# Autodesk Inventor assembly: switchback
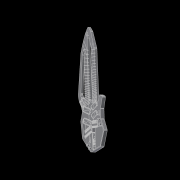
[picture p0: Inventor's stored thumbnail of the model, 180x180]
Saved by Autodesk Inventor 2020 (Build 240168000, 168)
## iProperties
Created: 2020-01-02
Part Number: switchback
Document SubType Name: Assembly
Designer: valer
Author: valer
## Documents named in this file (17)
- C:\Users\valer\Desktop\switchback\switchback.iam
- C:\Users\valer\Desktop\switchback\switchback.ipt
- C:\Users\valer\Desktop\switchback\strandberg-headless-tuner.ipt
- C:\Users\valer\Desktop\switchback\fishman-modern6.ipt
- C:\Users\valer\Desktop\switchback\fishman-modern8.ipt
- C:\Users\valer\Desktop\switchback\fishman-pot.ipt
- C:\Users\valer\Desktop\switchback\fishman-switch.ipt
- C:\Users\valer\Desktop\switchback\fishman-battery.ipt
- C:\Users\valer\Desktop\switchback\switchback-secondary-cover.ipt
- C:\Users\valer\Desktop\switchback\switchback-primary-cover.ipt
- C:\Users\valer\Desktop\switchback\fishman-jack.ipt
- C:\Users\valer\Desktop\switchback\switchback-pickup-cover-8.ipt
- C:\Users\valer\Desktop\switchback\switchback-pickup-cover-6.ipt
- C:\Users\valer\Desktop\switchback\switchback-logo-01.ipt
- C:\Users\valer\Desktop\switchback\arduino.ipt
- C:\Users\valer\Desktop\switchback\oscilloscope-screen.ipt
- C:\Users\valer\Desktop\switchback\switchback-osc-cover.ipt
## Components (38 placed, 16 different names)
1. switchback:1 — Mate:1, Mate:2, Tangent:1, Mate:4, Mate:5, Tangent:2, Mate:6, Mate:7, Tangent:3, Mate:8, Mate:9, Tangent:4, Mate:10, Mate:11, Tangent:5, Mate:12, Mate:13, Tangent:6, Mate:14, Mate:15, Tangent:7, Mate:16, Mate:17, Tangent:8, Mate:28, Mate:29, Tangent:14, Mate:42, Mate:43, Tangent:15, Mate:44, Mate:45, Tangent:16, Mate:46, Mate:47, Tangent:17, Mate:48, Mate:49, Tangent:18, Mate:50, Mate:51, Tangent:19, Mate:52, Mate:53, Mate:54, Mate:55, Mate:56, Mate:57, Mate:58, Mate:59, Mate:60, Mate:61, Mate:62, Mate:63, Mate:66, Mate:67, Mate:68, Mate:69, Mate:70, Mate:71, Mate:72, Mate:73, Angle:1, Angle:2, Angle:3, Angle:4, Mate:74, Mate:75, Mate:76, Mate:77, Mate:78, Mate:79, Mate:80, Mate:81, Mate:82, Mate:83, Mate:104, Mate:105, Mate:106, Mate:107, Mate:108, Mate:109, Flush:1, Mate:110, Mate:111, Mate:112, Mate:113, Mate:114, Mate:121, Mate:122
2. strandberg-headless-tuner:1 — Mate:1, Mate:2, Tangent:1
3. strandberg-headless-tuner:2 — Mate:4, Mate:5, Tangent:2
4. strandberg-headless-tuner:3 — Mate:6, Mate:7, Tangent:3
5. strandberg-headless-tuner:4 — Mate:10, Mate:11, Tangent:5
6. strandberg-headless-tuner:5 — Mate:12, Mate:13, Tangent:6
7. strandberg-headless-tuner:6 — Mate:8, Mate:9, Tangent:4
8. strandberg-headless-tuner:8 — Mate:14, Mate:15, Tangent:7
9. strandberg-headless-tuner:9 — Mate:16, Mate:17, Tangent:8
10. strandberg-headless-tuner:15 — Mate:28, Mate:29, Tangent:14
11. strandberg-headless-tuner:16 — Mate:46, Mate:47, Tangent:17
12. strandberg-headless-tuner:17 — Mate:48, Mate:49, Tangent:18
13. strandberg-headless-tuner:18 — Mate:42, Mate:43, Tangent:15
14. strandberg-headless-tuner:19 — Mate:44, Mate:45, Tangent:16
15. strandberg-headless-tuner:20 — Mate:50, Mate:51, Tangent:19
16. fishman-modern6:1 — Mate:52, Mate:53, Mate:54, Mate:101, Mate:102, Mate:103
17. fishman-modern6:2 — Mate:55, Mate:56, Mate:57, Mate:98, Mate:99, Mate:100
18. fishman-modern8:1 — Mate:61, Mate:62, Mate:63, Mate:92, Mate:95, Mate:96, Mate:97
19. fishman-modern8:2 — Mate:58, Mate:59, Mate:60, Mate:93, Mate:94
20. fishman-pot:1 — Mate:72, Mate:73, Angle:4
21. fishman-pot:2 — Mate:70, Mate:71, Angle:3
22. fishman-pot:4 — Mate:66, Mate:67, Angle:2
23. fishman-pot:5 — Mate:68, Mate:69, Angle:1
24. fishman-switch:1 — Mate:77, Mate:78, Mate:79
25. fishman-switch:2 — Mate:74, Mate:75, Mate:76
26. fishman-battery:1 — Mate:80, Mate:115, Mate:116, Angle:5
27. switchback-secondary-cover:1 — Mate:81, Mate:82, Mate:83
28. switchback-primary-cover:1 — Mate:115, Mate:116, Angle:5, Mate:117, Mate:118, Mate:119, Mate:120, Mate:121, Mate:122
29. fishman-jack:1 — Mate:118, Mate:119
30. fishman-jack:2 — Mate:117, Mate:120
31. switchback-pickup-cover-8:1 — Mate:92, Mate:93, Mate:94
32. switchback-pickup-cover-8:2 — Mate:95, Mate:96, Mate:97
33. switchback-pickup-cover-6:2 — Mate:98, Mate:99, Mate:100
34. switchback-pickup-cover-6:3 — Mate:101, Mate:102, Mate:103
35. switchback-logo-01:1 — Mate:104, Mate:105, Mate:106
36. arduino:1 — Mate:107, Mate:108, Mate:109
37. OscilloscopeScreen:1 — Flush:1, Mate:110, Mate:111
38. switchback-osc-cover:1 — Mate:112, Mate:113, Mate:114
## Relationships (109: Mate 89, Tangent 14, Angle 5, Flush 1)
- Mate:1: switchback:1 ↔ strandberg-headless-tuner:1
- Mate:2: switchback:1 ↔ strandberg-headless-tuner:1
- Tangent:1: switchback:1 ↔ strandberg-headless-tuner:1
- Mate:4: switchback:1 ↔ strandberg-headless-tuner:2
- Mate:5: switchback:1 ↔ strandberg-headless-tuner:2
- Tangent:2: switchback:1 ↔ strandberg-headless-tuner:2
- Mate:6: switchback:1 ↔ strandberg-headless-tuner:3
- Mate:7: switchback:1 ↔ strandberg-headless-tuner:3
- Tangent:3: switchback:1 ↔ strandberg-headless-tuner:3
- Mate:8: switchback:1 ↔ strandberg-headless-tuner:6
- Mate:9: switchback:1 ↔ strandberg-headless-tuner:6
- Tangent:4: switchback:1 ↔ strandberg-headless-tuner:6
- Mate:10: switchback:1 ↔ strandberg-headless-tuner:4
- Mate:11: switchback:1 ↔ strandberg-headless-tuner:4
- Tangent:5: switchback:1 ↔ strandberg-headless-tuner:4
- Mate:12: switchback:1 ↔ strandberg-headless-tuner:5
- Mate:13: switchback:1 ↔ strandberg-headless-tuner:5
- Tangent:6: switchback:1 ↔ strandberg-headless-tuner:5
- Mate:14: switchback:1 ↔ strandberg-headless-tuner:8
- Mate:15: switchback:1 ↔ strandberg-headless-tuner:8
- Tangent:7: switchback:1 ↔ strandberg-headless-tuner:8
- Mate:16: switchback:1 ↔ strandberg-headless-tuner:9
- Mate:17: switchback:1 ↔ strandberg-headless-tuner:9
- Tangent:8: switchback:1 ↔ strandberg-headless-tuner:9
- Mate:28: switchback:1 ↔ strandberg-headless-tuner:15
- Mate:29: switchback:1 ↔ strandberg-headless-tuner:15
- Tangent:14: switchback:1 ↔ strandberg-headless-tuner:15
- Mate:42: switchback:1 ↔ strandberg-headless-tuner:18
- Mate:43: switchback:1 ↔ strandberg-headless-tuner:18
- Tangent:15: switchback:1 ↔ strandberg-headless-tuner:18
- Mate:44: switchback:1 ↔ strandberg-headless-tuner:19
- Mate:45: switchback:1 ↔ strandberg-headless-tuner:19
- Tangent:16: switchback:1 ↔ strandberg-headless-tuner:19
- Mate:46: switchback:1 ↔ strandberg-headless-tuner:16
- Mate:47: switchback:1 ↔ strandberg-headless-tuner:16
- Tangent:17: switchback:1 ↔ strandberg-headless-tuner:16
- Mate:48: switchback:1 ↔ strandberg-headless-tuner:17
- Mate:49: switchback:1 ↔ strandberg-headless-tuner:17
- Tangent:18: switchback:1 ↔ strandberg-headless-tuner:17
- Mate:50: switchback:1 ↔ strandberg-headless-tuner:20
- Mate:51: switchback:1 ↔ strandberg-headless-tuner:20
- Tangent:19: switchback:1 ↔ strandberg-headless-tuner:20
- Mate:52: switchback:1 ↔ fishman-modern6:1
- Mate:53: switchback:1 ↔ fishman-modern6:1
- Mate:54: switchback:1 ↔ fishman-modern6:1
- Mate:55: switchback:1 ↔ fishman-modern6:2
- Mate:56: switchback:1 ↔ fishman-modern6:2
- Mate:57: switchback:1 ↔ fishman-modern6:2
- Mate:58: switchback:1 ↔ fishman-modern8:2
- Mate:59: switchback:1 ↔ fishman-modern8:2
- Mate:60: switchback:1 ↔ fishman-modern8:2
- Mate:61: switchback:1 ↔ fishman-modern8:1
- Mate:62: switchback:1 ↔ fishman-modern8:1
- Mate:63: switchback:1 ↔ fishman-modern8:1
- Mate:66: switchback:1 ↔ fishman-pot:4
- Mate:67: switchback:1 ↔ fishman-pot:4
- Mate:68: switchback:1 ↔ fishman-pot:5
- Mate:69: switchback:1 ↔ fishman-pot:5
- Mate:70: switchback:1 ↔ fishman-pot:2
- Mate:71: switchback:1 ↔ fishman-pot:2
- Mate:72: switchback:1 ↔ fishman-pot:1
- Mate:73: switchback:1 ↔ fishman-pot:1
- Angle:1 (180 deg): switchback:1 ↔ fishman-pot:5
- Angle:2 (180 deg): switchback:1 ↔ fishman-pot:4
- Angle:3 (180 deg): switchback:1 ↔ fishman-pot:2
- Angle:4 (180 deg): switchback:1 ↔ fishman-pot:1
- Mate:74: switchback:1 ↔ fishman-switch:2
- Mate:75: switchback:1 ↔ fishman-switch:2
- Mate:76: switchback:1 ↔ fishman-switch:2
- Mate:77: switchback:1 ↔ fishman-switch:1
- Mate:78: switchback:1 ↔ fishman-switch:1
- Mate:79: switchback:1 ↔ fishman-switch:1
- Mate:80: switchback:1 ↔ fishman-battery:1
- Mate:81: switchback:1 ↔ switchback-secondary-cover:1
- Mate:82: switchback:1 ↔ switchback-secondary-cover:1
- Mate:83: switchback:1 ↔ switchback-secondary-cover:1
- Mate:92: fishman-modern8:1 ↔ switchback-pickup-cover-8:1
- Mate:93: fishman-modern8:2 ↔ switchback-pickup-cover-8:1
- Mate:94: fishman-modern8:2 ↔ switchback-pickup-cover-8:1
- Mate:95: fishman-modern8:1 ↔ switchback-pickup-cover-8:2
- Mate:96: fishman-modern8:1 ↔ switchback-pickup-cover-8:2
- Mate:97: fishman-modern8:1 ↔ switchback-pickup-cover-8:2
- Mate:98: fishman-modern6:2 ↔ switchback-pickup-cover-6:2
- Mate:99: fishman-modern6:2 ↔ switchback-pickup-cover-6:2
- Mate:100: fishman-modern6:2 ↔ switchback-pickup-cover-6:2
- Mate:101: fishman-modern6:1 ↔ switchback-pickup-cover-6:3
- Mate:102: fishman-modern6:1 ↔ switchback-pickup-cover-6:3
- Mate:103: fishman-modern6:1 ↔ switchback-pickup-cover-6:3
- Mate:104: switchback:1 ↔ switchback-logo-01:1
- Mate:105: switchback:1 ↔ switchback-logo-01:1
- Mate:106: switchback:1 ↔ switchback-logo-01:1
- Mate:107: switchback:1 ↔ arduino:1
- Mate:108: switchback:1 ↔ arduino:1
- Mate:109: switchback:1 ↔ arduino:1
- Flush:1: switchback:1 ↔ OscilloscopeScreen:1
- Mate:110 (3.302 mm): switchback:1 ↔ OscilloscopeScreen:1
- Mate:111 (0.762 mm): switchback:1 ↔ OscilloscopeScreen:1
- Mate:112: switchback:1 ↔ switchback-osc-cover:1
- Mate:113: switchback:1 ↔ switchback-osc-cover:1
- Mate:114: switchback:1 ↔ switchback-osc-cover:1
- Mate:115: fishman-battery:1 ↔ switchback-primary-cover:1
- Mate:116: fishman-battery:1 ↔ switchback-primary-cover:1
- Angle:5 (0 deg): fishman-battery:1 ↔ switchback-primary-cover:1
- Mate:117: switchback-primary-cover:1 ↔ fishman-jack:2
- Mate:118: switchback-primary-cover:1 ↔ fishman-jack:1
- Mate:119: switchback-primary-cover:1 ↔ fishman-jack:1
- Mate:120: switchback-primary-cover:1 ↔ fishman-jack:2
- Mate:121: switchback:1 ↔ switchback-primary-cover:1
- Mate:122: switchback:1 ↔ switchback-primary-cover:1
